(part 1 of 2)
# Autodesk Inventor assembly: Prototype II Assembly V3
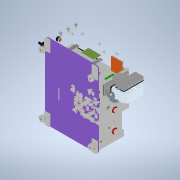
[picture p0: Inventor's stored thumbnail of the model, 180x180]
Saved by Autodesk Inventor 2021 (Build 250183000, 183)
## iProperties
Created: 2020-07-16
Part Number: Prototype II Assembly V3
Document SubType Name: Assembly
Designer: jgray
Author: jgray
## Documents named in this file (71)
- M:\Printed Electronics\Gas Sensors\Prototypes\Prototype II -Cartridge Reader V3\Prototype II Assembly V3.iam
- M:\Printed Electronics\Gas Sensors\Prototypes\Prototype II -Cartridge Reader V3\40ml Bottle and Lid.iam
- M:\Printed Electronics\Gas Sensors\Prototypes\Prototype II -Cartridge Reader V3\100ml Bottle and Lid.iam
- M:\Printed Electronics\Gas Sensors\Prototypes\Prototype II -Cartridge Reader V3\Full Cartridge Interface.iam
- M:\Printed Electronics\Gas Sensors\Prototypes\Prototype II -Cartridge Reader V3\Control & Sense Head PCB Assm.iam
- M:\Printed Electronics\Gas Sensors\Prototypes\Prototype II -Cartridge Reader V3\EC Sensor Sub-Assem.iam
- M:\Printed Electronics\Gas Sensors\Prototypes\Prototype II -Cartridge Reader V3\22Ah BatteryPack.ipt
- M:\Printed Electronics\Gas Sensors\Prototypes\Prototype II -Cartridge Reader V3\Battery Con.ipt
- M:\Printed Electronics\Gas Sensors\Prototypes\Prototype II -Cartridge Reader V3\Box Fixing Stud.ipt
- M:\Printed Electronics\Gas Sensors\Prototypes\Prototype II -Cartridge Reader V3\Coms Board V1.ipt
- M:\Printed Electronics\Gas Sensors\Prototypes\Prototype II -Cartridge Reader V3\Enclosure RS746-7396 body.ipt
- M:\Printed Electronics\Gas Sensors\Prototypes\Prototype II -Cartridge Reader V3\Internal Rear Plate.ipt
- M:\Printed Electronics\Gas Sensors\Prototypes\Prototype II -Cartridge Reader V3\Mechanical Driver Board.ipt
- M:\Printed Electronics\Gas Sensors\Prototypes\Prototype II -Cartridge Reader V3\Port Support Plate.ipt
- M:\Printed Electronics\Gas Sensors\Prototypes\Prototype II -Cartridge Reader V3\Right Bracket 50mm RS749-1680.ipt
- M:\Printed Electronics\Gas Sensors\Prototypes\Prototype II -Cartridge Reader V3\Status Indicator PCB.ipt
- M:\Printed Electronics\Gas Sensors\Prototypes\Prototype II -Cartridge Reader V3\Switch Mode PS PCB.ipt
- M:\Printed Electronics\Gas Sensors\Prototypes\Prototype II -Cartridge Reader V3\Top Divider.ipt
- M:\Printed Electronics\Gas Sensors\Prototypes\Prototype II -Cartridge Reader V3\Union Elbow 1-8 KQ2L01-00A SMC.ipt
- M:\Printed Electronics\Gas Sensors\Prototypes\Prototype II -Cartridge Reader V3\Vent Port M12.ipt
- M:\Printed Electronics\Gas Sensors\Prototypes\Prototype II -Cartridge Reader V3\Union Tee 1-8 KQ2T01-00A SMC.ipt
- M:\Printed Electronics\Gas Sensors\Prototypes\Prototype II -Cartridge Reader V3\Right Bracket 30mm RS749-1686.ipt
- M:\Printed Electronics\Gas Sensors\Prototypes\Prototype II -Cartridge Reader V3\Mounted Pump.iam
- M:\Printed Electronics\Gas Sensors\Prototypes\Prototype II -Cartridge Reader V3\Valve Assembly.iam
- M:\Printed Electronics\Gas Sensors\Prototypes\Prototype II -Cartridge Reader V3\Inner Top Plate.ipt
- M:\Printed Electronics\Gas Sensors\Prototypes\Prototype II -Cartridge Reader V3\Battery Side Plate.ipt
- M:\Printed Electronics\Gas Sensors\Prototypes\Prototype II -Cartridge Reader V3\LED Indicator Assem Farnell 1368996.iam
- M:\Printed Electronics\Gas Sensors\Prototypes\Prototype II -Cartridge Reader V3\Omron Switch DigiKey_Z6183-NDA22NS_2B[]_N[]A_G[]00_NN.iam
- M:\Printed Electronics\Gas Sensors\Prototypes\Prototype II -Cartridge Reader V3\Sprung Button Assm DigiKey EG5980-ND.iam
- M:\Printed Electronics\Gas Sensors\Prototypes\Prototype II -Cartridge Reader V3\Fixing Stud Pt 2.ipt
- M:\Printed Electronics\Gas Sensors\Prototypes\Prototype II -Cartridge Reader V3\Port Conversion Nut.ipt
- M:\Printed Electronics\Gas Sensors\Prototypes\Prototype II -Cartridge Reader V3\M8 Mudguard Washer RS 660-4771.ipt
- M:\Printed Electronics\Gas Sensors\Prototypes\Prototype II -Cartridge Reader V3\M12 Form B A2 Washer RS 530-810.ipt
- M:\Printed Electronics\Gas Sensors\Prototypes\Prototype II -Cartridge Reader V3\M12 Tap washer RS 530-270.ipt
- M:\Printed Electronics\Gas Sensors\Prototypes\Prototype II -Cartridge Reader V3\Cable Gland Lock Nut RS 822-9791.ipt
- M:\Printed Electronics\Gas Sensors\Prototypes\Prototype II -Cartridge Reader V3\SMC AS2002F Needle Valve RS 827-0755.ipt
- M:\Printed Electronics\Gas Sensors\Prototypes\Prototype II -Cartridge Reader V3\Battery Base Plate.ipt
- M:\Printed Electronics\Gas Sensors\Prototypes\Prototype II -Cartridge Reader V3\Internal Vert Divider.ipt
- M:\Printed Electronics\Gas Sensors\Prototypes\Prototype II -Cartridge Reader V3\SMC10-32UNF-1-8 KQ2H01-32N RS 840-4665.ipt
- M:\Printed Electronics\Gas Sensors\Prototypes\Prototype II -Cartridge Reader V3\Tube 1-8 5L.ipt
- M:\Printed Electronics\Gas Sensors\Prototypes\Prototype II -Cartridge Reader V3\SMC Elbow KQ2L23-04.ipt
- M:\Printed Electronics\Gas Sensors\Prototypes\Prototype II -Cartridge Reader V3\Legris4-4mm Elbow 31820400 RS 306-5993.ipt
- M:\Printed Electronics\Gas Sensors\Prototypes\Prototype II -Cartridge Reader V3\SMC Nipple 1-8to5-32 KQ2N01-03.ipt
- M:\Printed Electronics\Gas Sensors\Prototypes\Prototype II -Cartridge Reader V3\SMC 4mmMale-1-8Push KQ2R01-03(R23-04).ipt
- M:\Printed Electronics\Gas Sensors\Prototypes\Prototype II -Cartridge Reader V3\Bottle Base Plate.ipt
- M:\Printed Electronics\Gas Sensors\Prototypes\Prototype II -Cartridge Reader V3\Single Thrd Right Support Farnell1466883.ipt
- M:\Printed Electronics\Gas Sensors\Prototypes\Prototype II -Cartridge Reader V3\No Thrd Right Support Farnell1466881.ipt
- M:\Printed Electronics\Gas Sensors\Prototypes\Prototype II -Cartridge Reader V3\Cable Clip 3-1Dia RS817-8956.ipt
- M:\Printed Electronics\Gas Sensors\Prototypes\Prototype II -Cartridge Reader V3\Door Lock.ipt
- M:\Printed Electronics\Gas Sensors\Prototypes\Prototype II -Cartridge Reader V3\BAttery divider.ipt
- M:\Printed Electronics\Gas Sensors\Prototypes\Prototype II -Cartridge Reader V3\Bottle side plate.ipt
- M:\Printed Electronics\Gas Sensors\Prototypes\Prototype II -Cartridge Reader V3\Battery Top Plate.ipt
- C:\Users\jgray\Documents\Inventor\Content Center Files\R2021\en-US\BS 4320(2)\BS 4320 - M8 (Form B).ipt
- C:\Users\jgray\Documents\Inventor\Content Center Files\R2021\en-US\DIN 934\DIN 934 - M8 x 1.25.ipt
- M:\Printed Electronics\Gas Sensors\Prototypes\Prototype II -Cartridge Reader V3\Bottle Spacer Base.ipt
- M:\Printed Electronics\Gas Sensors\Prototypes\Prototype II -Cartridge Reader V3\Lower slide.ipt
- M:\Printed Electronics\Gas Sensors\Prototypes\Prototype II -Cartridge Reader V3\Upper slide.ipt
- M:\Printed Electronics\Gas Sensors\Prototypes\Prototype II -Cartridge Reader V3\Gas Side Top Cover.ipt
- M:\Printed Electronics\Gas Sensors\Prototypes\Prototype II -Cartridge Reader V3\Battery Cover.ipt
- M:\Printed Electronics\Gas Sensors\Prototypes\Prototype II -Cartridge Reader V3\Electronics cover.ipt
- M:\Printed Electronics\Gas Sensors\Prototypes\Prototype II -Cartridge Reader V3\corner spacers.ipt
- M:\Printed Electronics\Gas Sensors\Prototypes\Prototype II -Cartridge Reader V3\Silicone Seal washer.ipt
- M:\Printed Electronics\Gas Sensors\Prototypes\Prototype II -Cartridge Reader V3\Step-back spacer -electronics enc.ipt
- M:\Printed Electronics\Gas Sensors\Prototypes\Prototype II -Cartridge Reader V3\Step-back cover -electronics enc.ipt
- M:\Printed Electronics\Gas Sensors\Prototypes\Prototype II -Cartridge Reader V3\Top Bottle Front.ipt
- M:\Printed Electronics\Gas Sensors\Prototypes\Prototype II -Cartridge Reader V3\Top Bottle Middle.ipt
- M:\Printed Electronics\Gas Sensors\Prototypes\Prototype II -Cartridge Reader V3\Top Bottle Back.ipt
- M:\Printed Electronics\Gas Sensors\Prototypes\Prototype II -Cartridge Reader V3\upper plate slide.ipt
- M:\Printed Electronics\Gas Sensors\Prototypes\Prototype II -Cartridge Reader V3\LiPo cover.ipt
- M:\Printed Electronics\Gas Sensors\Prototypes\Prototype II -Cartridge Reader V3\Lipo Battery.ipt
- M:\Printed Electronics\Gas Sensors\Prototypes\Prototype II -Cartridge Reader V3\LipoBat Spacer.ipt
## Components (233 placed, 70 different names)
1. 40ml Bottle and Lid:1 [sub-assembly] — Angle:10, Mate:46, Mate:47, Mate:60, Mate:61, Flush:20, Flush:21, Flush:22
2. 40ml Bottle and Lid:2 [sub-assembly] — Angle:9, Mate:44, Mate:45, Mate:62, Mate:63, Flush:22
3. 40ml Bottle and Lid:3 [sub-assembly] — Angle:8, Mate:52, Mate:53, Mate:54, Mate:55, Flush:21
4. 40ml Bottle and Lid:4 [sub-assembly] — Angle:7, Mate:58, Flush:20, Flush:23, Mate:371
5. 100ml Bottle and Lid:1 [sub-assembly] — Angle:6, Mate:56, Flush:23, Mate:268
6. Full Cartridge Interface:1 [sub-assembly] — Mate:7, Mate:8, Mate:9, Mate:14, Mate:229, Mate:230, Mate:231, Mate:232, Flush:29, Mate:346, Flush:30
7. Control & Sense Head PCB Assm:1 [sub-assembly] — Flush:29, Mate:346, Flush:30
8. EC Sensor Sub-Assem:1 [sub-assembly] — Angle:1, Angle:2, Mate:12, Flush:8
9. 22Ah BatteryPack:1 — Mate:2, Mate:67, Flush:14, Mate:415, Mate:416, Mate:417
10. 22Ah BatteryPack:2 — Mate:1, Flush:14, Mate:145, Mate:383, Mate:622
11. Battery Con:1 — Mate:622
12. Battery Con:2 — Mate:415, Angle:66, Mate:416, Mate:417
13. Box Fixing Stud:1 — Mate:31, Mate:32, Mate:97, Mate:98, Mate:521, Mate:527, Mate:614
14. Box Fixing Stud:2 — Mate:35, Flush:11, Mate:102, Mate:517, Mate:525, Mate:610, Mate:615
15. Box Fixing Stud:3 — Mate:36, Flush:10, Mate:99, Mate:101, Angle:67, Mate:513, Mate:514, Mate:612, Mate:616
16. Box Fixing Stud:4 — Mate:33, Mate:34, Flush:10, Flush:11, Mate:6, Mate:100, Mate:519, Mate:526, Mate:619
17. Coms Board V1:1 — Mate:629, Mate:630, Mate:631, Mate:636, Mate:637, Mate:675
18. Enclosure RS746-7396 body:1 — Mate:5, Mate:7, Mate:8, Mate:9, Mate:13, Mate:15, Mate:31, Mate:32, Mate:33, Mate:34, Mate:35, Mate:36, Mate:78, Mate:79, Mate:80, Mate:81, Mate:82, Mate:83, Mate:84, Mate:85, Mate:86, Mate:87, Mate:88, Mate:89, Mate:90, Flush:15, Mate:91, Mate:92, Mate:94, Mate:96, Mate:105, Mate:106, Mate:107, Mate:108, Mate:113, Mate:114, Mate:122, Tangent:1, Tangent:2, Tangent:3, Tangent:4
19. Internal Rear Plate:1 — Mate:1, Mate:2, Mate:5, Mate:6, Angle:1, Angle:2, Mate:12, Angle:3, Angle:4, Flush:8, Mate:22, Angle:5, Mate:24, Flush:9, Mate:25, Mate:26, Mate:27, Mate:28, Mate:29, Mate:30, Mate:41, Mate:43, Mate:65, Mate:72, Mate:74, Mate:124, Mate:125, Mate:126, Mate:127, Mate:128, Mate:129, Mate:130, Mate:133, Mate:139, Mate:140, Mate:141, Angle:16, Angle:17, Angle:18, Angle:21, Mate:174, Angle:22, Angle:24, Mate:177, Mate:178, Mate:182, Mate:183, Angle:27, Angle:29, Mate:186, Mate:191, Mate:196, Mate:197, Mate:199, Angle:35, Angle:36, Angle:38, Mate:210, Mate:69, Mate:221, Mate:222, Mate:224, Mate:227, Angle:48, Mate:235, Mate:238, Angle:53, Mate:257, Mate:269, Mate:270, Mate:273, Mate:274, Angle:56, Angle:57, Angle:58, Mate:292, Mate:313, Mate:314, Mate:340, Mate:341, Mate:342, Mate:343, Mate:344, Mate:348, Mate:349, Mate:350, Mate:352, Mate:353, Mate:354, Mate:364, Angle:60, Angle:61, Angle:62, Angle:63, Angle:64, Angle:65, Mate:386, Mate:392, Mate:393, Mate:394, Mate:412, Mate:414, Mate:423, Mate:446, Mate:449, Mate:465, Mate:467, Mate:468, Mate:469, Mate:470, Mate:486, Mate:487, Mate:500, Mate:502, Mate:507, Mate:511, Mate:512, Mate:516, Mate:518, Mate:520, Mate:528, Mate:607, Mate:609, Mate:611, Angle:80, Mate:613, Angle:81, Mate:648, Mate:661, Mate:664
20. Mechanical Driver Board:1 — Mate:375, Mate:378, Mate:379
21. Port Support Plate:1 — Mate:13, Mate:14, Mate:15, Mate:16, Mate:17, Mate:18, Mate:19, Mate:20, Mate:21, Mate:70, Flush:31, Mate:375, Mate:378, Mate:379
22. Right Bracket 50mm RS749-1680:1 — Mate:25, Mate:26, Mate:27, Mate:75, Mate:77
23. Right Bracket 50mm RS749-1680:2 — Mate:28, Mate:29, Mate:30, Mate:76
24. Right Bracket 50mm RS749-1680:3 — Mate:72, Mate:73, Mate:74
25. Right Bracket 50mm RS749-1680:4 — Mate:16, Mate:18, Mate:19, Mate:23
26. Right Bracket 50mm RS749-1680:5 — Mate:17, Mate:20, Mate:21
27. Status Indicator PCB:1 — Mate:670, Mate:671, Mate:672
28. Switch Mode PS PCB:1 — Mate:22, Angle:5, Mate:344
29. Top Divider:1 — Mate:23, Mate:24, Flush:9, Mate:40, Flush:13, Mate:66, Mate:73, Angle:14, Angle:45, Angle:46, Angle:47, Mate:233, Mate:244, Mate:374, Mate:376, Mate:377, Mate:388, Mate:389, Mate:390, Mate:397, Mate:399, Mate:418, Mate:421, Mate:551, Flush:33, Flush:34, Mate:553, Mate:554, Mate:556, Mate:557, Mate:580, Mate:581, Flush:45, Flush:46, Mate:583, Mate:584, Mate:591, Mate:592, Angle:72, Angle:73, Angle:74, Angle:75, Mate:594, Mate:595, Mate:596, Mate:603, Mate:604, Mate:605, Angle:77, Angle:78, Angle:79, Mate:632, Mate:633, Mate:634, Mate:635, Mate:673, Mate:676, Mate:678, Mate:679, Mate:680, Mate:681
30. Union Elbow 1-8 KQ2L01-00A SMC:1 — Angle:22, Mate:182, Mate:185, Flush:24, Angle:27, Mate:192, Mate:194, Mate:322, Mate:323
31. Vent Port M12:1 — Mate:78, Mate:82, Mate:103, Mate:116
32. Union Elbow 1-8 KQ2L01-00A SMC:2 — Mate:178, Mate:337, Mate:338, Mate:339
33. Vent Port M12:2 — Mate:79, Mate:81, Mate:123
34. Union Elbow 1-8 KQ2L01-00A SMC:3 — Flush:16, Angle:18
35. Union Elbow 1-8 KQ2L01-00A SMC:4 — Mate:56, Flush:16, Mate:211
36. Union Elbow 1-8 KQ2L01-00A SMC:5 — Mate:53, Mate:55, Flush:18, Mate:184, Angle:28, Angle:32
37. Union Elbow 1-8 KQ2L01-00A SMC:6 — Mate:52, Mate:54, Flush:18, Angle:16, Mate:181
38. Union Elbow 1-8 KQ2L01-00A SMC:7 — Mate:223, Angle:60, Mate:371
39. Union Elbow 1-8 KQ2L01-00A SMC:8 — Mate:58, Mate:372
40. Union Elbow 1-8 KQ2L01-00A SMC:9 — Mate:46, Mate:61, Angle:23, Mate:176, Mate:256
41. Union Elbow 1-8 KQ2L01-00A SMC:10 — Mate:47, Mate:60, Mate:187, Mate:370
42. Union Elbow 1-8 KQ2L01-00A SMC:11 — Mate:45, Mate:62, Flush:17, Mate:337
43. Union Elbow 1-8 KQ2L01-00A SMC:12 — Mate:44, Mate:63, Flush:17, Angle:17, Mate:185
44. Union Tee 1-8 KQ2T01-00A SMC:1 — Mate:239, Mate:240, Angle:50, Mate:241, Angle:55, Mate:313, Mate:353
45. Union Tee 1-8 KQ2T01-00A SMC:2 — Angle:29, Mate:186, Mate:187, Mate:189, Mate:190, Mate:204, Mate:332, Mate:333, Angle:64, Mate:370
46. Union Tee 1-8 KQ2T01-00A SMC:3 — Angle:21, Mate:174, Mate:181, Mate:204, Angle:38, Mate:330, Mate:334
47. Right Bracket 30mm RS749-1686:2 — Mate:408, Mate:409, Mate:410, Mate:411
48. Right Bracket 30mm RS749-1686:3 — Mate:404, Mate:405, Mate:406, Mate:407
49. Right Bracket 30mm RS749-1686:4 — Mate:401, Mate:402, Mate:403
50. Right Bracket 30mm RS749-1686:5 — Mate:397, Mate:398, Mate:399, Mate:400
51. Right Bracket 30mm RS749-1686:6 — Mate:388, Mate:389, Mate:390, Mate:391
52. Right Bracket 30mm RS749-1686:8 — Mate:253, Mate:254, Mate:255, Angle:54
53. Mounted Pump:1 [sub-assembly] — Mate:70, Flush:31, Mate:374
54. Valve Assembly:1 [sub-assembly] — Mate:69, Angle:40, Mate:342
55. Valve Assembly:2 [sub-assembly] — Mate:196, Angle:34, Mate:340
56. Valve Assembly:3 [sub-assembly] — Mate:191, Angle:32, Angle:34, Angle:40, Mate:341
57. Inner Top Plate:1 — Mate:75, Mate:76, Mate:77, Mate:598, Mate:599, Mate:623, Mate:624, Mate:625, Mate:626, Mate:627, Mate:667, Mate:668, Mate:669, Mate:670, Mate:671, Mate:672
58. Right Bracket 50mm RS749-1680:8 — Mate:40, Mate:41, Mate:43
59. Battery Side Plate:1 — Mate:65, Flush:13, Mate:66, Mate:67, Mate:131, Mate:132, Mate:134, Mate:135, Mate:404, Mate:406, Mate:419, Mate:420, Mate:464, Mate:471, Mate:490, Mate:558, Mate:574, Mate:575, Flush:42, Mate:579, Flush:47
60. Vent Port M12:3 — Mate:80, Mate:83, Mate:104, Mate:115, Mate:119
61. LED Indicator Assem Farnell 1368996:1 [sub-assembly] — Mate:84, Mate:89
62. LED Indicator Assem Farnell 1368996:2 [sub-assembly] — Mate:86, Mate:87
63. LED Indicator Assem Farnell 1368996:3 [sub-assembly] — Mate:85, Mate:88
64. Omron Switch DigiKey_Z6183-NDA22NS_2B[]_N[]A_G[]00_NN:1 [sub-assembly] — Mate:90, Flush:15, Angle:14
65. Sprung Button Assm DigiKey EG5980-ND:1 [sub-assembly] — Mate:91, Mate:92
66. Fixing Stud Pt 2:1 — Mate:94, Mate:100, Mate:111, Mate:608, Mate:620
67. Fixing Stud Pt 2:2 — Mate:99, Mate:101, Mate:109, Mate:618
68. Fixing Stud Pt 2:3 — Mate:96, Mate:102, Mate:110, Mate:617
69. Fixing Stud Pt 2:4 — Mate:97, Mate:98, Mate:112, Mate:621
70. Port Conversion Nut:1 — Mate:103, Mate:121, Mate:157, Mate:159, Mate:160
71. Port Conversion Nut:2 — Mate:104, Mate:120, Mate:158, Mate:161
72. M8 Mudguard Washer RS 660-4771:1 — Mate:107, Mate:112
73. M8 Mudguard Washer RS 660-4771:2 — Mate:105, Mate:111
74. M8 Mudguard Washer RS 660-4771:3 — Mate:108, Mate:109
75. M8 Mudguard Washer RS 660-4771:4 — Mate:106, Mate:110
76. M12 Form B A2 Washer RS 530-810:1 — Mate:117, Mate:121, Mate:157
77. M12 Tap washer RS 530-270:1 — Mate:113, Mate:116, Mate:117
78. M12 Form B A2 Washer RS 530-810:2 — Mate:118, Mate:119, Mate:120
79. M12 Tap washer RS 530-270:2 — Mate:114, Mate:115, Mate:118
80. Cable Gland Lock Nut RS 822-9791:1 — Mate:122, Mate:123
81. Right Bracket 50mm RS749-1680:9 — Mate:133, Mate:134, Mate:135
82. Right Bracket 50mm RS749-1680:10 — Mate:130, Mate:131, Mate:132
83. Right Bracket 50mm RS749-1680:12 — Mate:392, Mate:393, Mate:394, Mate:395, Mate:396
84. Right Bracket 50mm RS749-1680:13 — Mate:139, Mate:140, Mate:141, Mate:142, Mate:143, Mate:144
85. SMC AS2002F Needle Valve RS 827-0755:1 — Mate:244, Mate:246, Flush:28, Mate:248, Mate:252, Mate:376, Mate:377
86. Right Bracket 50mm RS749-1680:14 — Mate:125, Mate:128, Mate:129, Mate:137, Mate:138
87. Right Bracket 50mm RS749-1680:15 — Mate:507, Mate:508, Mate:509, Mate:510, Mate:511
88. Right Bracket 50mm RS749-1680:17 — Mate:124, Mate:126, Mate:127, Mate:136
89. Battery Base Plate:1 — Mate:136, Mate:137, Mate:138, Mate:145, Mate:384, Mate:385, Mate:401, Mate:403, Mate:405, Mate:407, Mate:408, Mate:411, Mate:564, Mate:565, Mate:566, Mate:567, Mate:569, Mate:570, Mate:571, Mate:572, Flush:37, Flush:38, Flush:39, Flush:40
90. Internal Vert Divider:1 — Mate:142, Mate:143, Mate:144, Mate:255, Mate:258, Mate:271, Mate:272, Mate:383, Mate:387, Mate:391, Mate:409, Mate:410, Mate:413, Mate:459, Mate:461, Mate:462, Mate:497, Mate:498, Mate:505, Mate:506, Mate:529, Mate:531, Mate:533, Mate:539, Mate:540, Mate:541, Mate:548, Mate:549, Flush:35, Mate:561, Mate:562, Mate:573, Flush:36, Mate:577, Mate:585, Mate:586, Mate:587, Mate:588, Mate:589, Mate:590, Mate:647, Mate:662, Mate:665, Mate:666, Mate:677
91. SMC10-32UNF-1-8 KQ2H01-32N RS 840-4665:1 — Mate:159, Mate:160, Mate:163, Mate:164, Mate:251
92. SMC10-32UNF-1-8 KQ2H01-32N RS 840-4665:2 — Mate:158, Mate:161, Mate:345
93. Tube 1-8 5L:2 — Mate:163, Mate:164
94. Union Elbow 1-8 KQ2L01-00A SMC:14 — Mate:171, Angle:23, Angle:24, Mate:176, Mate:256
95. Union Elbow 1-8 KQ2L01-00A SMC:15 — Mate:171, Mate:345
96. Union Elbow 1-8 KQ2L01-00A SMC:16 — Mate:189, Mate:190, Mate:209
97. Union Elbow 1-8 KQ2L01-00A SMC:17 — Mate:197, Mate:201, Angle:35, Angle:39, Mate:315, Mate:316, Mate:348, Angle:63, Angle:65
98. Union Elbow 1-8 KQ2L01-00A SMC:18 — Mate:177, Mate:192, Mate:194, Mate:309, Mate:310
99. Union Elbow 1-8 KQ2L01-00A SMC:19 — Mate:199, Mate:202, Mate:203, Angle:49, Mate:295, Mate:296, Mate:350
100. Union Elbow 1-8 KQ2L01-00A SMC:20 — Mate:183, Mate:184, Flush:24, Angle:28, Mate:193, Mate:195, Flush:25, Angle:44
101. Union Elbow 1-8 KQ2L01-00A SMC:21 — Mate:193, Mate:195, Flush:25, Mate:318, Mate:319
102. Union Elbow 1-8 KQ2L01-00A SMC:22 — Mate:201, Mate:202, Mate:203, Angle:36, Angle:37, Mate:207, Mate:354
103. Union Elbow 1-8 KQ2L01-00A SMC:23 — Mate:210, Mate:211, Angle:39, Mate:277, Mate:328, Mate:329, Mate:349
104. Union Elbow 1-8 KQ2L01-00A SMC:24 — Mate:208, Mate:209
105. Union Elbow 1-8 KQ2L01-00A SMC:26 — Angle:37, Mate:207, Mate:208, Mate:290, Mate:291, Mate:292
106. Union Elbow 1-8 KQ2L01-00A SMC:28 — Mate:221, Mate:226, Angle:53, Angle:55, Mate:282, Mate:283, Mate:284, Mate:285
107. Union Elbow 1-8 KQ2L01-00A SMC:29 — Mate:222, Mate:223, Mate:226, Angle:44, Angle:51, Mate:326, Mate:327, Mate:364, Angle:62
108. Union Elbow 1-8 KQ2L01-00A SMC:30 — Mate:224, Angle:50, Angle:51, Mate:314, Mate:324, Mate:325, Angle:61, Mate:372
109. Union Elbow 1-8 KQ2L01-00A SMC:31 — Mate:227, Mate:277, Mate:303, Mate:304, Mate:305, Mate:306, Mate:343
110. Union Elbow 1-8 KQ2L01-00A SMC:32 — Mate:251, Mate:253, Mate:254, Angle:54
111. SMC Elbow KQ2L23-04:2 — Mate:248, Mate:252
112. Legris4-4mm Elbow 31820400 RS 306-5993:1 — Mate:231, Mate:232, Angle:45, Mate:243, Flush:27
113. Legris4-4mm Elbow 31820400 RS 306-5993:2 — Mate:229, Mate:230, Angle:46, Mate:234, Mate:242, Flush:26
114. Union Elbow 1-8 KQ2L01-00A SMC:33 — Mate:235, Mate:236, Angle:49, Mate:241, Mate:299, Mate:300, Mate:301, Mate:302
115. Union Elbow 1-8 KQ2L01-00A SMC:34 — Angle:47, Angle:48, Mate:233, Mate:234, Mate:236
116. Union Elbow 1-8 KQ2L01-00A SMC:35 — Mate:238, Mate:239, Mate:240, Mate:278, Mate:279, Mate:280, Mate:281
117. SMC Nipple 1-8to5-32 KQ2N01-03:1 — Mate:243, Flush:27
118. SMC Nipple 1-8to5-32 KQ2N01-03:2 — Mate:246, Flush:28
119. SMC 4mmMale-1-8Push KQ2R01-03(R23-04):2 — Mate:242, Flush:26
120. Bottle Base Plate:1 — Mate:257, Mate:258, Mate:268, Mate:275, Mate:276, Mate:422, Mate:424, Flush:32, Mate:450, Mate:451, Mate:453, Mate:454, Mate:456, Mate:457, Mate:458, Mate:460, Mate:463, Angle:67, Mate:530, Mate:532, Mate:535
121. Single Thrd Right Support Farnell1466883:8 — Mate:565, Mate:571, Flush:38
122. No Thrd Right Support Farnell1466881:1 — Mate:269, Mate:273, Mate:275
123. No Thrd Right Support Farnell1466881:2 — Mate:270, Mate:274, Mate:276
124. No Thrd Right Support Farnell1466881:3 — Mate:271, Mate:387
125. No Thrd Right Support Farnell1466881:4 — Mate:448, Mate:454, Mate:455, Mate:457
126. No Thrd Right Support Farnell1466881:5 — Mate:447, Mate:452, Mate:453, Mate:456
127. No Thrd Right Support Farnell1466881:6 — Mate:446, Mate:449, Mate:450, Mate:451
128. No Thrd Right Support Farnell1466881:7 — Mate:468, Mate:496, Mate:501, Mate:502
129. No Thrd Right Support Farnell1466881:8 — Mate:470, Mate:479, Mate:485, Mate:486
130. No Thrd Right Support Farnell1466881:9 — Mate:272, Mate:422, Mate:458, Mate:459
131. No Thrd Right Support Farnell1466881:11 — Mate:469, Mate:478, Mate:487, Mate:488
132. No Thrd Right Support Farnell1466881:12 — Mate:467, Mate:495, Mate:499, Mate:500
133. Cable Clip 3-1Dia RS817-8956:2 — Angle:56, Mate:278, Mate:281
134. Cable Clip 3-1Dia RS817-8956:3 — Angle:58, Mate:330, Mate:334
135. Cable Clip 3-1Dia RS817-8956:4 — Angle:57, Mate:279, Mate:280
136. Cable Clip 3-1Dia RS817-8956:5 — Mate:282, Mate:285
137. Cable Clip 3-1Dia RS817-8956:6 — Mate:283, Mate:284
138. Cable Clip 3-1Dia RS817-8956:9 — Mate:290, Mate:291
139. Cable Clip 3-1Dia RS817-8956:12 — Mate:295, Mate:296
140. Cable Clip 3-1Dia RS817-8956:13 — Mate:299, Mate:300
141. Cable Clip 3-1Dia RS817-8956:14 — Mate:301, Mate:302
142. Cable Clip 3-1Dia RS817-8956:15 — Mate:303, Mate:304
143. Cable Clip 3-1Dia RS817-8956:16 — Mate:305, Mate:306
144. Cable Clip 3-1Dia RS817-8956:19 — Mate:322, Mate:323
145. Cable Clip 3-1Dia RS817-8956:20 — Mate:328, Mate:329, Mate:352
146. Cable Clip 3-1Dia RS817-8956:22 — Mate:309, Mate:310
147. Cable Clip 3-1Dia RS817-8956:24 — Mate:318, Mate:319
148. Cable Clip 3-1Dia RS817-8956:25 — Mate:315, Mate:316
149. Cable Clip 3-1Dia RS817-8956:26 — Mate:324, Mate:325
150. Cable Clip 3-1Dia RS817-8956:27 — Mate:326, Mate:327
151. Cable Clip 3-1Dia RS817-8956:29 — Mate:332, Mate:333
152. Cable Clip 3-1Dia RS817-8956:30 — Mate:338, Mate:339
153. Door Lock:1 — Tangent:3, Tangent:4
154. Door Lock:2 — Tangent:1, Tangent:2
155. BAttery divider:1 — Mate:384, Mate:385, Mate:386, Mate:395, Mate:396, Mate:398, Mate:400, Mate:402, Angle:66, Mate:466, Mate:480, Mate:481, Mate:484, Mate:491, Mate:493, Mate:494, Mate:563, Mate:568, Flush:41
156. Right Bracket 30mm RS749-1686:9 — Mate:412, Mate:413, Mate:414
157. Right Bracket 30mm RS749-1686:10 — Mate:418, Mate:419, Mate:420, Mate:421
158. Bottle side plate:1 — Mate:423, Mate:424, Flush:32, Mate:447, Mate:448, Mate:452, Mate:455, Mate:508, Mate:509, Mate:510, Mate:536, Mate:537, Mate:538, Mate:542, Mate:543, Mate:544, Mate:545, Mate:546, Mate:552, Mate:582, Mate:593, Angle:71, Mate:650, Mate:654, Mate:659
159. Single Thrd Right Support Farnell1466883:9 — Mate:548, Mate:549, Angle:69, Mate:550
160. Single Thrd Right Support Farnell1466883:10 — Mate:557, Mate:580, Flush:46
161. Single Thrd Right Support Farnell1466883:13 — Mate:545, Mate:546, Angle:68, Mate:547
162. Single Thrd Right Support Farnell1466883:15 — Mate:556, Mate:581, Flush:45
163. Single Thrd Right Support Farnell1466883:16 — Mate:558, Mate:579, Flush:47
164. Single Thrd Right Support Farnell1466883:17 — Mate:559, Mate:578, Flush:44
165. Single Thrd Right Support Farnell1466883:18 — Mate:560, Mate:576, Flush:43
166. Single Thrd Right Support Farnell1466883:19 — Mate:561, Mate:577, Angle:70
167. No Thrd Right Support Farnell1466881:13 — Mate:460, Mate:461, Mate:462, Mate:463
168. Battery Top Plate:1 — Mate:464, Mate:465, Mate:466, Mate:472, Mate:473, Mate:474, Mate:475, Mate:476, Mate:477, Mate:478, Mate:479, Mate:482, Mate:483, Mate:485, Mate:488, Mate:489, Mate:492, Mate:495, Mate:496, Mate:499, Mate:501, Mate:503, Mate:504, Mate:559, Mate:560, Mate:576, Mate:578, Flush:43, Flush:44, Angle:70
169. No Thrd Right Support Farnell1466881:16 — Mate:476, Mate:498, Mate:504, Mate:505
170. No Thrd Right Support Farnell1466881:17 — Mate:474, Mate:492, Mate:493, Mate:494
171. No Thrd Right Support Farnell1466881:18 — Mate:473, Mate:481, Mate:482, Mate:491
172. No Thrd Right Support Farnell1466881:19 — Mate:471, Mate:477, Mate:489, Mate:490
173. No Thrd Right Support Farnell1466881:20 — Mate:472, Mate:480, Mate:483, Mate:484
174. No Thrd Right Support Farnell1466881:21 — Mate:475, Mate:497, Mate:503, Mate:506
175. BS 4320 Form AB M8 (Form B):1 — Mate:512, Mate:513, Mate:515
176. BS 4320 Form AB M8 (Form B):2 — Mate:516, Mate:517, Mate:524
177. BS 4320 Form AB M8 (Form B):3 — Mate:520, Mate:521, Mate:522
178. BS 4320 Form AB M8 (Form B):4 — Mate:518, Mate:519, Mate:523
179. DIN 934 - replaced by DIN EN 24032/28673/28674 M8:1 — Mate:524, Mate:525
180. DIN 934 - replaced by DIN EN 24032/28673/28674 M8:2 — Mate:514, Mate:515
181. DIN 934 - replaced by DIN EN 24032/28673/28674 M8:3 — Mate:522, Mate:527
182. DIN 934 - replaced by DIN EN 24032/28673/28674 M8:4 — Mate:523, Mate:526
183. Bottle Spacer Base:1 — Mate:528, Mate:529, Mate:530, Angle:68, Mate:547, Angle:69, Mate:550
184. Lower slide:1 — Mate:535, Mate:536, Mate:537, Mate:538
185. Lower slide:2 — Mate:531, Mate:532, Mate:533, Mate:677
186. Upper slide:1 — Mate:542, Mate:543, Mate:544, Mate:646, Mate:655, Mate:658
187. Upper slide:2 — Mate:539, Mate:540, Mate:541, Mate:649, Mate:652, Mate:656, Mate:657
188. Gas Side Top Cover:1 — Mate:551, Mate:552, Flush:33
189. Battery Cover:1 — Flush:34, Flush:35, Mate:553
190. Electronics cover:1 — Mate:554, Mate:638, Mate:639, Mate:640, Mate:641, Mate:642
191. Single Thrd Right Support Farnell1466883:20 — Mate:563, Mate:568, Flush:41
192. Single Thrd Right Support Farnell1466883:21 — Mate:564, Mate:572, Flush:37
193. Single Thrd Right Support Farnell1466883:22 — Mate:567, Mate:570, Flush:40
194. Single Thrd Right Support Farnell1466883:23 — Mate:586, Mate:589, Angle:75, Angle:76
195. Single Thrd Right Support Farnell1466883:24 — Mate:587, Mate:588, Angle:76
196. Single Thrd Right Support Farnell1466883:25 — Mate:562, Mate:573, Flush:36
197. Single Thrd Right Support Farnell1466883:26 — Mate:566, Mate:569, Flush:39
198. Single Thrd Right Support Farnell1466883:27 — Mate:582, Mate:593, Angle:71
199. Single Thrd Right Support Farnell1466883:28 — Mate:583, Mate:592, Angle:72
200. Single Thrd Right Support Farnell1466883:29 — Mate:584, Mate:591, Angle:73
201. Single Thrd Right Support Farnell1466883:31 — Mate:585, Mate:590, Angle:74
202. Single Thrd Right Support Farnell1466883:32 — Mate:574, Mate:575, Flush:42
203. Single Thrd Right Support Farnell1466883:33 — Mate:594, Mate:603, Angle:79, Mate:638, Mate:639
204. Single Thrd Right Support Farnell1466883:34 — Mate:595, Mate:604, Angle:78
205. Single Thrd Right Support Farnell1466883:35 — Mate:599, Mate:667
206. Single Thrd Right Support Farnell1466883:36 — Mate:596, Mate:605, Angle:77
207. Single Thrd Right Support Farnell1466883:37 — Mate:598, Mate:669
208. corner spacers:1 — Mate:613, Mate:614, Angle:81
209. corner spacers:2 — Mate:611, Mate:612, Angle:80
210. corner spacers:3 — Mate:609, Mate:610
211. corner spacers:4 — Mate:607, Mate:608
212. Silicone Seal washer:1 — Mate:621
213. Silicone Seal washer:2 — Mate:619, Mate:620
214. Silicone Seal washer:3 — Mate:615, Mate:617
215. Silicone Seal washer:4 — Mate:616, Mate:618
216. Single Thrd Right Support Farnell1466883:38 — Mate:625, Mate:626, Mate:630
217. Single Thrd Right Support Farnell1466883:39 — Mate:632, Mate:633, Mate:636, Mate:675
218. Single Thrd Right Support Farnell1466883:40 — Mate:627, Mate:668
219. Single Thrd Right Support Farnell1466883:41 — Mate:623, Mate:624, Mate:629, Mate:631
220. Single Thrd Right Support Farnell1466883:42 — Mate:634, Mate:635, Mate:637
221. Step-back spacer -electronics enc:1 — Mate:640, Mate:641, Mate:642, Mate:643, Mate:644, Mate:645
222. Step-back cover -electronics enc:1 — Mate:643, Mate:644, Mate:645
223. Top Bottle Front:1 — Mate:652, Mate:653, Mate:654, Angle:82, Angle:83
224. Top Bottle Middle:1 — Mate:649, Mate:650, Mate:651, Mate:653, Mate:660, Mate:663
225. Top Bottle Back:1 — Mate:646, Mate:647, Mate:648, Mate:651
226. Single Thrd Right Support Farnell1466883:43 — Mate:655, Mate:658, Angle:82
227. Single Thrd Right Support Farnell1466883:44 — Mate:656, Mate:657, Angle:83
228. upper plate slide:1 — Mate:659, Mate:660, Mate:661
229. upper plate slide:2 — Mate:662, Mate:663, Mate:664, Mate:665, Mate:666
230. LiPo cover:1 — Mate:673, Flush:48
231. Lipo Battery:1 — Mate:676, Flush:48
232. LipoBat Spacer:1 — Mate:679, Mate:680, Mate:681, Mate:682, Flush:50
233. LipoBat Spacer:2 — Mate:678, Mate:682, Flush:50
## Relationships (653: Mate 542, Angle 67, Flush 40, Tangent 4)
- Mate:1: 22Ah BatteryPack:2 ↔ Internal Rear Plate:1
- Mate:2: 22Ah BatteryPack:1 ↔ Internal Rear Plate:1
- Mate:5 (0.6 mm): Enclosure RS746-7396 body:1 ↔ Internal Rear Plate:1
- Mate:6: Box Fixing Stud:4 ↔ Internal Rear Plate:1
- Mate:7: Full Cartridge Interface:1 ↔ Enclosure RS746-7396 body:1
- Mate:8: Full Cartridge Interface:1 ↔ Enclosure RS746-7396 body:1
- Mate:9: Full Cartridge Interface:1 ↔ Enclosure RS746-7396 body:1
- Angle:1 (180 deg): EC Sensor Sub-Assem:1 ↔ Internal Rear Plate:1
- Angle:2 (0 deg): EC Sensor Sub-Assem:1 ↔ Internal Rear Plate:1
- Mate:12 (2 mm): EC Sensor Sub-Assem:1 ↔ Internal Rear Plate:1
- Angle:3 (180 deg): Internal Rear Plate:1
- Angle:4 (180 deg): Internal Rear Plate:1
- Flush:8 (40 mm): EC Sensor Sub-Assem:1 ↔ Internal Rear Plate:1
- Mate:13: Enclosure RS746-7396 body:1 ↔ Port Support Plate:1
- Mate:14: Full Cartridge Interface:1 ↔ Port Support Plate:1
- Mate:15: Enclosure RS746-7396 body:1 ↔ Port Support Plate:1
- Mate:16: Port Support Plate:1 ↔ Right Bracket 50mm RS749-1680:4
- Mate:17: Port Support Plate:1 ↔ Right Bracket 50mm RS749-1680:5
- Mate:18: Port Support Plate:1 ↔ Right Bracket 50mm RS749-1680:4
- Mate:19: Port Support Plate:1 ↔ Right Bracket 50mm RS749-1680:4
- Mate:20: Port Support Plate:1 ↔ Right Bracket 50mm RS749-1680:5
- Mate:21: Port Support Plate:1 ↔ Right Bracket 50mm RS749-1680:5
- Mate:22 (8 mm): Internal Rear Plate:1 ↔ Switch Mode PS PCB:1
- Angle:5 (90 deg): Internal Rear Plate:1 ↔ Switch Mode PS PCB:1
- Angle:6 (0 deg): 100ml Bottle and Lid:1
- Angle:7 (0 deg): 40ml Bottle and Lid:4
- Angle:8 (0 deg): 40ml Bottle and Lid:3
- Angle:9 (0 deg): 40ml Bottle and Lid:2
- Angle:10 (0 deg): 40ml Bottle and Lid:1
- Mate:23: Right Bracket 50mm RS749-1680:4 ↔ Top Divider:1
- Mate:24: Internal Rear Plate:1 ↔ Top Divider:1
- Flush:9: Internal Rear Plate:1 ↔ Top Divider:1
- Mate:25: Internal Rear Plate:1 ↔ Right Bracket 50mm RS749-1680:1
- Mate:26: Internal Rear Plate:1 ↔ Right Bracket 50mm RS749-1680:1
- Mate:27: Internal Rear Plate:1 ↔ Right Bracket 50mm RS749-1680:1
- Mate:28: Internal Rear Plate:1 ↔ Right Bracket 50mm RS749-1680:2
- Mate:29: Internal Rear Plate:1 ↔ Right Bracket 50mm RS749-1680:2
- Mate:30: Internal Rear Plate:1 ↔ Right Bracket 50mm RS749-1680:2
- Mate:31: Box Fixing Stud:1 ↔ Enclosure RS746-7396 body:1
- Mate:32 (1 mm): Box Fixing Stud:1 ↔ Enclosure RS746-7396 body:1
- Mate:33: Box Fixing Stud:4 ↔ Enclosure RS746-7396 body:1
- Mate:34 (1 mm): Box Fixing Stud:4 ↔ Enclosure RS746-7396 body:1
- Mate:35: Box Fixing Stud:2 ↔ Enclosure RS746-7396 body:1
- Mate:36: Box Fixing Stud:3 ↔ Enclosure RS746-7396 body:1
- Flush:10: Box Fixing Stud:3 ↔ Box Fixing Stud:4
- Flush:11: Box Fixing Stud:2 ↔ Box Fixing Stud:4
- Mate:40: Top Divider:1 ↔ Right Bracket 50mm RS749-1680:8
- Mate:41: Internal Rear Plate:1 ↔ Right Bracket 50mm RS749-1680:8
- Mate:43: Internal Rear Plate:1 ↔ Right Bracket 50mm RS749-1680:8
- Mate:44 (8 mm): 40ml Bottle and Lid:2 ↔ Union Elbow 1-8 KQ2L01-00A SMC:12
- Mate:45: 40ml Bottle and Lid:2 ↔ Union Elbow 1-8 KQ2L01-00A SMC:11
- Mate:46: 40ml Bottle and Lid:1 ↔ Union Elbow 1-8 KQ2L01-00A SMC:9
- Mate:47: 40ml Bottle and Lid:1 ↔ Union Elbow 1-8 KQ2L01-00A SMC:10
- Mate:52: 40ml Bottle and Lid:3 ↔ Union Elbow 1-8 KQ2L01-00A SMC:6
- Mate:53 (8 mm): 40ml Bottle and Lid:3 ↔ Union Elbow 1-8 KQ2L01-00A SMC:5
- Mate:54: 40ml Bottle and Lid:3 ↔ Union Elbow 1-8 KQ2L01-00A SMC:6
- Mate:55: 40ml Bottle and Lid:3 ↔ Union Elbow 1-8 KQ2L01-00A SMC:5
- Mate:56: 100ml Bottle and Lid:1 ↔ Union Elbow 1-8 KQ2L01-00A SMC:4
- Mate:58: 40ml Bottle and Lid:4 ↔ Union Elbow 1-8 KQ2L01-00A SMC:8
- Mate:60: 40ml Bottle and Lid:1 ↔ Union Elbow 1-8 KQ2L01-00A SMC:10
- Mate:61: 40ml Bottle and Lid:1 ↔ Union Elbow 1-8 KQ2L01-00A SMC:9
- Mate:62: 40ml Bottle and Lid:2 ↔ Union Elbow 1-8 KQ2L01-00A SMC:11
- Mate:63: 40ml Bottle and Lid:2 ↔ Union Elbow 1-8 KQ2L01-00A SMC:12
- Mate:65: Internal Rear Plate:1 ↔ Battery Side Plate:1
- Flush:13: Top Divider:1 ↔ Battery Side Plate:1
- Mate:66: Top Divider:1 ↔ Battery Side Plate:1
- Mate:67 (0.1 mm): 22Ah BatteryPack:1 ↔ Battery Side Plate:1
- Flush:14: 22Ah BatteryPack:1 ↔ 22Ah BatteryPack:2
- Mate:69: Internal Rear Plate:1 ↔ Valve Assembly:1
- Mate:70: Port Support Plate:1 ↔ Mounted Pump:1
- Mate:72: Internal Rear Plate:1 ↔ Right Bracket 50mm RS749-1680:3
- Mate:73: Right Bracket 50mm RS749-1680:3 ↔ Top Divider:1
- Mate:74: Internal Rear Plate:1 ↔ Right Bracket 50mm RS749-1680:3
- Mate:75: Right Bracket 50mm RS749-1680:1 ↔ Inner Top Plate:1
- Mate:76: Right Bracket 50mm RS749-1680:2 ↔ Inner Top Plate:1
- Mate:77: Right Bracket 50mm RS749-1680:1 ↔ Inner Top Plate:1
- Mate:78: Enclosure RS746-7396 body:1 ↔ Vent Port M12:1
- Mate:79: Enclosure RS746-7396 body:1 ↔ Vent Port M12:2
- Mate:80: Enclosure RS746-7396 body:1 ↔ Vent Port M12:3
- Mate:81 (1 mm): Enclosure RS746-7396 body:1 ↔ Vent Port M12:2
- Mate:82 (1 mm): Enclosure RS746-7396 body:1 ↔ Vent Port M12:1
- Mate:83 (1 mm): Enclosure RS746-7396 body:1 ↔ Vent Port M12:3
- Mate:84: Enclosure RS746-7396 body:1 ↔ LED Indicator Assem Farnell 1368996:1
- Mate:85: Enclosure RS746-7396 body:1 ↔ LED Indicator Assem Farnell 1368996:3
- Mate:86: Enclosure RS746-7396 body:1 ↔ LED Indicator Assem Farnell 1368996:2
- Mate:87: Enclosure RS746-7396 body:1 ↔ LED Indicator Assem Farnell 1368996:2
- Mate:88: Enclosure RS746-7396 body:1 ↔ LED Indicator Assem Farnell 1368996:3
- Mate:89: Enclosure RS746-7396 body:1 ↔ LED Indicator Assem Farnell 1368996:1
- Mate:90: Enclosure RS746-7396 body:1 ↔ Omron Switch DigiKey_Z6183-NDA22NS_2B[]_N[]A_G[]00_NN:1
- Flush:15: Enclosure RS746-7396 body:1 ↔ Omron Switch DigiKey_Z6183-NDA22NS_2B[]_N[]A_G[]00_NN:1
- Angle:14 (0 deg): Top Divider:1 ↔ Omron Switch DigiKey_Z6183-NDA22NS_2B[]_N[]A_G[]00_NN:1
- Mate:91: Enclosure RS746-7396 body:1 ↔ Sprung Button Assm DigiKey EG5980-ND:1
- Mate:92: Enclosure RS746-7396 body:1 ↔ Sprung Button Assm DigiKey EG5980-ND:1
- Mate:94: Enclosure RS746-7396 body:1 ↔ Fixing Stud Pt 2:1
- Mate:96: Enclosure RS746-7396 body:1 ↔ Fixing Stud Pt 2:3
- Mate:97: Box Fixing Stud:1 ↔ Fixing Stud Pt 2:4
- Mate:98: Box Fixing Stud:1 ↔ Fixing Stud Pt 2:4
- Mate:99: Box Fixing Stud:3 ↔ Fixing Stud Pt 2:2
- Mate:100: Box Fixing Stud:4 ↔ Fixing Stud Pt 2:1
- Mate:101: Box Fixing Stud:3 ↔ Fixing Stud Pt 2:2
- Mate:102: Box Fixing Stud:2 ↔ Fixing Stud Pt 2:3
- Mate:103: Vent Port M12:1 ↔ Port Conversion Nut:1
- Mate:104: Vent Port M12:3 ↔ Port Conversion Nut:2
- Mate:105: Enclosure RS746-7396 body:1 ↔ M8 Mudguard Washer RS 660-4771:2
- Mate:106: Enclosure RS746-7396 body:1 ↔ M8 Mudguard Washer RS 660-4771:4
- Mate:107: Enclosure RS746-7396 body:1 ↔ M8 Mudguard Washer RS 660-4771:1
- Mate:108: Enclosure RS746-7396 body:1 ↔ M8 Mudguard Washer RS 660-4771:3
- Mate:109: Fixing Stud Pt 2:2 ↔ M8 Mudguard Washer RS 660-4771:3
- Mate:110: Fixing Stud Pt 2:3 ↔ M8 Mudguard Washer RS 660-4771:4
- Mate:111: Fixing Stud Pt 2:1 ↔ M8 Mudguard Washer RS 660-4771:2
- Mate:112: Fixing Stud Pt 2:4 ↔ M8 Mudguard Washer RS 660-4771:1
- Mate:113: Enclosure RS746-7396 body:1 ↔ M12 Tap washer RS 530-270:1
- Mate:114: Enclosure RS746-7396 body:1 ↔ M12 Tap washer RS 530-270:2
- Mate:115: Vent Port M12:3 ↔ M12 Tap washer RS 530-270:2
- Mate:116: Vent Port M12:1 ↔ M12 Tap washer RS 530-270:1
- Mate:117: M12 Form B A2 Washer RS 530-810:1 ↔ M12 Tap washer RS 530-270:1
- Mate:118: M12 Form B A2 Washer RS 530-810:2 ↔ M12 Tap washer RS 530-270:2
- Mate:119: Vent Port M12:3 ↔ M12 Form B A2 Washer RS 530-810:2
- Mate:120: Port Conversion Nut:2 ↔ M12 Form B A2 Washer RS 530-810:2
- Mate:121: Port Conversion Nut:1 ↔ M12 Form B A2 Washer RS 530-810:1
- Mate:122: Enclosure RS746-7396 body:1 ↔ Cable Gland Lock Nut RS 822-9791:1
- Mate:123: Vent Port M12:2 ↔ Cable Gland Lock Nut RS 822-9791:1
- Mate:124: Internal Rear Plate:1 ↔ Right Bracket 50mm RS749-1680:17
- Mate:125: Internal Rear Plate:1 ↔ Right Bracket 50mm RS749-1680:14
- Mate:126: Internal Rear Plate:1 ↔ Right Bracket 50mm RS749-1680:17
- Mate:127: Internal Rear Plate:1 ↔ Right Bracket 50mm RS749-1680:17
- Mate:128: Internal Rear Plate:1 ↔ Right Bracket 50mm RS749-1680:14
- Mate:129: Internal Rear Plate:1 ↔ Right Bracket 50mm RS749-1680:14
- Mate:130: Internal Rear Plate:1 ↔ Right Bracket 50mm RS749-1680:10
- Mate:131: Battery Side Plate:1 ↔ Right Bracket 50mm RS749-1680:10
- Mate:132: Battery Side Plate:1 ↔ Right Bracket 50mm RS749-1680:10
- Mate:133: Internal Rear Plate:1 ↔ Right Bracket 50mm RS749-1680:9
- Mate:134: Battery Side Plate:1 ↔ Right Bracket 50mm RS749-1680:9
- Mate:135: Battery Side Plate:1 ↔ Right Bracket 50mm RS749-1680:9
- Mate:136: Right Bracket 50mm RS749-1680:17 ↔ Battery Base Plate:1
- Mate:137: Right Bracket 50mm RS749-1680:14 ↔ Battery Base Plate:1
- Mate:138: Right Bracket 50mm RS749-1680:14 ↔ Battery Base Plate:1
- Mate:139: Internal Rear Plate:1 ↔ Right Bracket 50mm RS749-1680:13
- Mate:140: Internal Rear Plate:1 ↔ Right Bracket 50mm RS749-1680:13
- Mate:141: Internal Rear Plate:1 ↔ Right Bracket 50mm RS749-1680:13
- Mate:142: Right Bracket 50mm RS749-1680:13 ↔ Internal Vert Divider:1
- Mate:143: Right Bracket 50mm RS749-1680:13 ↔ Internal Vert Divider:1
- Mate:144: Right Bracket 50mm RS749-1680:13 ↔ Internal Vert Divider:1
- Mate:145: 22Ah BatteryPack:2 ↔ Battery Base Plate:1
- Flush:16: Union Elbow 1-8 KQ2L01-00A SMC:3 ↔ Union Elbow 1-8 KQ2L01-00A SMC:4
- Flush:17: Union Elbow 1-8 KQ2L01-00A SMC:11 ↔ Union Elbow 1-8 KQ2L01-00A SMC:12
- Flush:18: Union Elbow 1-8 KQ2L01-00A SMC:5 ↔ Union Elbow 1-8 KQ2L01-00A SMC:6
- Mate:157: Port Conversion Nut:1 ↔ M12 Form B A2 Washer RS 530-810:1
- Angle:16 (-90 deg): Internal Rear Plate:1 ↔ Union Elbow 1-8 KQ2L01-00A SMC:6
- Angle:17 (-90 deg): Internal Rear Plate:1 ↔ Union Elbow 1-8 KQ2L01-00A SMC:12
- Angle:18 (90 deg): Internal Rear Plate:1 ↔ Union Elbow 1-8 KQ2L01-00A SMC:3
- Mate:158: Port Conversion Nut:2 ↔ SMC10-32UNF-1-8 KQ2H01-32N RS 840-4665:2
- Mate:159: Port Conversion Nut:1 ↔ SMC10-32UNF-1-8 KQ2H01-32N RS 840-4665:1
- Mate:160: Port Conversion Nut:1 ↔ SMC10-32UNF-1-8 KQ2H01-32N RS 840-4665:1
- Mate:161: Port Conversion Nut:2 ↔ SMC10-32UNF-1-8 KQ2H01-32N RS 840-4665:2
- Mate:163: SMC10-32UNF-1-8 KQ2H01-32N RS 840-4665:1 ↔ Tube 1-8 5L:2
- Mate:164: SMC10-32UNF-1-8 KQ2H01-32N RS 840-4665:1 ↔ Tube 1-8 5L:2
- Mate:171: Union Elbow 1-8 KQ2L01-00A SMC:14 ↔ Union Elbow 1-8 KQ2L01-00A SMC:15
- Angle:21 (0 deg): Internal Rear Plate:1 ↔ Union Tee 1-8 KQ2T01-00A SMC:3
- Mate:174: Internal Rear Plate:1 ↔ Union Tee 1-8 KQ2T01-00A SMC:3
- Flush:20: 40ml Bottle and Lid:1 ↔ 40ml Bottle and Lid:4
- Flush:21: 40ml Bottle and Lid:1 ↔ 40ml Bottle and Lid:3
- Flush:22: 40ml Bottle and Lid:1 ↔ 40ml Bottle and Lid:2
- Angle:22 (0 deg): Internal Rear Plate:1 ↔ Union Elbow 1-8 KQ2L01-00A SMC:1
- Angle:23 (180 deg): Union Elbow 1-8 KQ2L01-00A SMC:9 ↔ Union Elbow 1-8 KQ2L01-00A SMC:14
- Angle:24 (180 deg): Internal Rear Plate:1 ↔ Union Elbow 1-8 KQ2L01-00A SMC:14
- Mate:176: Union Elbow 1-8 KQ2L01-00A SMC:9 ↔ Union Elbow 1-8 KQ2L01-00A SMC:14
- Mate:177: Internal Rear Plate:1 ↔ Union Elbow 1-8 KQ2L01-00A SMC:18
- Mate:178: Internal Rear Plate:1 ↔ Union Elbow 1-8 KQ2L01-00A SMC:2
- Mate:181: Union Elbow 1-8 KQ2L01-00A SMC:6 ↔ Union Tee 1-8 KQ2T01-00A SMC:3
- Flush:23: 40ml Bottle and Lid:4 ↔ 100ml Bottle and Lid:1
- Mate:182: Internal Rear Plate:1 ↔ Union Elbow 1-8 KQ2L01-00A SMC:1
- Mate:183: Internal Rear Plate:1 ↔ Union Elbow 1-8 KQ2L01-00A SMC:20
- Mate:184: Union Elbow 1-8 KQ2L01-00A SMC:5 ↔ Union Elbow 1-8 KQ2L01-00A SMC:20
- Mate:185: Union Elbow 1-8 KQ2L01-00A SMC:1 ↔ Union Elbow 1-8 KQ2L01-00A SMC:12
- Flush:24: Union Elbow 1-8 KQ2L01-00A SMC:1 ↔ Union Elbow 1-8 KQ2L01-00A SMC:20
- Angle:27 (0 deg): Internal Rear Plate:1 ↔ Union Elbow 1-8 KQ2L01-00A SMC:1
- Angle:28 (180 deg): Union Elbow 1-8 KQ2L01-00A SMC:5 ↔ Union Elbow 1-8 KQ2L01-00A SMC:20
- Angle:29 (0 deg): Internal Rear Plate:1 ↔ Union Tee 1-8 KQ2T01-00A SMC:2
- Mate:186: Internal Rear Plate:1 ↔ Union Tee 1-8 KQ2T01-00A SMC:2
- Mate:187: Union Elbow 1-8 KQ2L01-00A SMC:10 ↔ Union Tee 1-8 KQ2T01-00A SMC:2
- Mate:189: Union Tee 1-8 KQ2T01-00A SMC:2 ↔ Union Elbow 1-8 KQ2L01-00A SMC:16
- Mate:190 (5 mm): Union Tee 1-8 KQ2T01-00A SMC:2 ↔ Union Elbow 1-8 KQ2L01-00A SMC:16
- Mate:191: Internal Rear Plate:1 ↔ Valve Assembly:3
- Angle:32 (0 deg): Union Elbow 1-8 KQ2L01-00A SMC:5 ↔ Valve Assembly:3
- Mate:192 (5 mm): Union Elbow 1-8 KQ2L01-00A SMC:1 ↔ Union Elbow 1-8 KQ2L01-00A SMC:18
- Mate:193 (5 mm): Union Elbow 1-8 KQ2L01-00A SMC:20 ↔ Union Elbow 1-8 KQ2L01-00A SMC:21
- Mate:194: Union Elbow 1-8 KQ2L01-00A SMC:1 ↔ Union Elbow 1-8 KQ2L01-00A SMC:18
- Mate:195: Union Elbow 1-8 KQ2L01-00A SMC:20 ↔ Union Elbow 1-8 KQ2L01-00A SMC:21
- Mate:196: Internal Rear Plate:1 ↔ Valve Assembly:2
- Mate:197: Internal Rear Plate:1 ↔ Union Elbow 1-8 KQ2L01-00A SMC:17
- Angle:34 (180 deg): Valve Assembly:2 ↔ Valve Assembly:3
- Mate:199: Internal Rear Plate:1 ↔ Union Elbow 1-8 KQ2L01-00A SMC:19
- Mate:201: Union Elbow 1-8 KQ2L01-00A SMC:17 ↔ Union Elbow 1-8 KQ2L01-00A SMC:22
- Mate:202 (4 mm): Union Elbow 1-8 KQ2L01-00A SMC:19 ↔ Union Elbow 1-8 KQ2L01-00A SMC:22
- Mate:203: Union Elbow 1-8 KQ2L01-00A SMC:19 ↔ Union Elbow 1-8 KQ2L01-00A SMC:22
- Mate:204: Union Tee 1-8 KQ2T01-00A SMC:2 ↔ Union Tee 1-8 KQ2T01-00A SMC:3
- Flush:25: Union Elbow 1-8 KQ2L01-00A SMC:20 ↔ Union Elbow 1-8 KQ2L01-00A SMC:21
- Angle:35 (0 deg): Internal Rear Plate:1 ↔ Union Elbow 1-8 KQ2L01-00A SMC:17
- Angle:36 (180 deg): Internal Rear Plate:1 ↔ Union Elbow 1-8 KQ2L01-00A SMC:22
- Angle:37 (0 deg): Union Elbow 1-8 KQ2L01-00A SMC:22 ↔ Union Elbow 1-8 KQ2L01-00A SMC:26
- Mate:207: Union Elbow 1-8 KQ2L01-00A SMC:22 ↔ Union Elbow 1-8 KQ2L01-00A SMC:26
- Mate:208: Union Elbow 1-8 KQ2L01-00A SMC:24 ↔ Union Elbow 1-8 KQ2L01-00A SMC:26
- Mate:209: Union Elbow 1-8 KQ2L01-00A SMC:16 ↔ Union Elbow 1-8 KQ2L01-00A SMC:24
- Angle:38 (0 deg): Internal Rear Plate:1 ↔ Union Tee 1-8 KQ2T01-00A SMC:3
- Mate:210: Internal Rear Plate:1 ↔ Union Elbow 1-8 KQ2L01-00A SMC:23
- Mate:211: Union Elbow 1-8 KQ2L01-00A SMC:4 ↔ Union Elbow 1-8 KQ2L01-00A SMC:23
- Angle:39 (0 deg): Union Elbow 1-8 KQ2L01-00A SMC:17 ↔ Union Elbow 1-8 KQ2L01-00A SMC:23
- Angle:40 (0 deg): Valve Assembly:1 ↔ Valve Assembly:3
- Mate:221: Internal Rear Plate:1 ↔ Union Elbow 1-8 KQ2L01-00A SMC:28
- Mate:222: Internal Rear Plate:1 ↔ Union Elbow 1-8 KQ2L01-00A SMC:29
- Mate:223: Union Elbow 1-8 KQ2L01-00A SMC:7 ↔ Union Elbow 1-8 KQ2L01-00A SMC:29
- Mate:224: Internal Rear Plate:1 ↔ Union Elbow 1-8 KQ2L01-00A SMC:30
- Mate:226 (75 mm): Union Elbow 1-8 KQ2L01-00A SMC:28 ↔ Union Elbow 1-8 KQ2L01-00A SMC:29
- Angle:44 (0 deg): Union Elbow 1-8 KQ2L01-00A SMC:20 ↔ Union Elbow 1-8 KQ2L01-00A SMC:29
- Mate:227: Internal Rear Plate:1 ↔ Union Elbow 1-8 KQ2L01-00A SMC:31
- Mate:229: Full Cartridge Interface:1 ↔ Legris4-4mm Elbow 31820400 RS 306-5993:2
- Mate:230: Full Cartridge Interface:1 ↔ Legris4-4mm Elbow 31820400 RS 306-5993:2
- Mate:231: Full Cartridge Interface:1 ↔ Legris4-4mm Elbow 31820400 RS 306-5993:1
- Mate:232: Full Cartridge Interface:1 ↔ Legris4-4mm Elbow 31820400 RS 306-5993:1
- Angle:45 (180 deg): Top Divider:1 ↔ Legris4-4mm Elbow 31820400 RS 306-5993:1
- Angle:46 (180 deg): Top Divider:1 ↔ Legris4-4mm Elbow 31820400 RS 306-5993:2
- Angle:47 (180 deg): Top Divider:1 ↔ Union Elbow 1-8 KQ2L01-00A SMC:34
- Angle:48 (180 deg): Internal Rear Plate:1 ↔ Union Elbow 1-8 KQ2L01-00A SMC:34
- Mate:233 (30 mm): Top Divider:1 ↔ Union Elbow 1-8 KQ2L01-00A SMC:34
- Mate:234: Legris4-4mm Elbow 31820400 RS 306-5993:2 ↔ Union Elbow 1-8 KQ2L01-00A SMC:34
- Mate:235: Internal Rear Plate:1 ↔ Union Elbow 1-8 KQ2L01-00A SMC:33
- Mate:236: Union Elbow 1-8 KQ2L01-00A SMC:33 ↔ Union Elbow 1-8 KQ2L01-00A SMC:34
- Angle:49 (0 deg): Union Elbow 1-8 KQ2L01-00A SMC:19 ↔ Union Elbow 1-8 KQ2L01-00A SMC:33
- Mate:238: Internal Rear Plate:1 ↔ Union Elbow 1-8 KQ2L01-00A SMC:35
- Mate:239 (48 mm): Union Tee 1-8 KQ2T01-00A SMC:1 ↔ Union Elbow 1-8 KQ2L01-00A SMC:35
- Mate:240: Union Tee 1-8 KQ2T01-00A SMC:1 ↔ Union Elbow 1-8 KQ2L01-00A SMC:35
- Angle:50 (180 deg): Union Tee 1-8 KQ2T01-00A SMC:1 ↔ Union Elbow 1-8 KQ2L01-00A SMC:30
- Angle:51 (0 deg): Union Elbow 1-8 KQ2L01-00A SMC:29 ↔ Union Elbow 1-8 KQ2L01-00A SMC:30
- Mate:241: Union Tee 1-8 KQ2T01-00A SMC:1 ↔ Union Elbow 1-8 KQ2L01-00A SMC:33
- Mate:242: Legris4-4mm Elbow 31820400 RS 306-5993:2 ↔ SMC 4mmMale-1-8Push KQ2R01-03(R23-04):2
- Flush:26 (-18 mm): Legris4-4mm Elbow 31820400 RS 306-5993:2 ↔ SMC 4mmMale-1-8Push KQ2R01-03(R23-04):2
- Mate:243: Legris4-4mm Elbow 31820400 RS 306-5993:1 ↔ SMC Nipple 1-8to5-32 KQ2N01-03:1
- Flush:27 (26.5 mm): Legris4-4mm Elbow 31820400 RS 306-5993:1 ↔ SMC Nipple 1-8to5-32 KQ2N01-03:1
- Mate:244 (15 mm): Top Divider:1 ↔ SMC AS2002F Needle Valve RS 827-0755:1
- Mate:246: SMC AS2002F Needle Valve RS 827-0755:1 ↔ SMC Nipple 1-8to5-32 KQ2N01-03:2
- Flush:28 (-26 mm): SMC AS2002F Needle Valve RS 827-0755:1 ↔ SMC Nipple 1-8to5-32 KQ2N01-03:2
- Mate:248 (-10 mm): SMC AS2002F Needle Valve RS 827-0755:1 ↔ SMC Elbow KQ2L23-04:2
- Mate:251: SMC10-32UNF-1-8 KQ2H01-32N RS 840-4665:1 ↔ Union Elbow 1-8 KQ2L01-00A SMC:32
- Mate:252: SMC AS2002F Needle Valve RS 827-0755:1 ↔ SMC Elbow KQ2L23-04:2
- Mate:253: Right Bracket 30mm RS749-1686:8 ↔ Union Elbow 1-8 KQ2L01-00A SMC:32
- Mate:254: Right Bracket 30mm RS749-1686:8 ↔ Union Elbow 1-8 KQ2L01-00A SMC:32
- Mate:255: Right Bracket 30mm RS749-1686:8 ↔ Internal Vert Divider:1
- Angle:53 (0 deg): Internal Rear Plate:1 ↔ Union Elbow 1-8 KQ2L01-00A SMC:28
- Mate:256 (34 mm): Union Elbow 1-8 KQ2L01-00A SMC:9 ↔ Union Elbow 1-8 KQ2L01-00A SMC:14
- Mate:257: Internal Rear Plate:1 ↔ Bottle Base Plate:1
- Mate:258: Internal Vert Divider:1 ↔ Bottle Base Plate:1
- Mate:268: 100ml Bottle and Lid:1 ↔ Bottle Base Plate:1
- Mate:269: Internal Rear Plate:1 ↔ No Thrd Right Support Farnell1466881:1
- Mate:270: Internal Rear Plate:1 ↔ No Thrd Right Support Farnell1466881:2
- Mate:271: Internal Vert Divider:1 ↔ No Thrd Right Support Farnell1466881:3
- Mate:272: Internal Vert Divider:1 ↔ No Thrd Right Support Farnell1466881:9
- Mate:273: Internal Rear Plate:1 ↔ No Thrd Right Support Farnell1466881:1
- Mate:274: Internal Rear Plate:1 ↔ No Thrd Right Support Farnell1466881:2
- Mate:275: Bottle Base Plate:1 ↔ No Thrd Right Support Farnell1466881:1
- Mate:276: Bottle Base Plate:1 ↔ No Thrd Right Support Farnell1466881:2
- Angle:54 (0 deg): Right Bracket 30mm RS749-1686:8 ↔ Union Elbow 1-8 KQ2L01-00A SMC:32
- Mate:277: Union Elbow 1-8 KQ2L01-00A SMC:23 ↔ Union Elbow 1-8 KQ2L01-00A SMC:31
- Angle:55 (0 deg): Union Tee 1-8 KQ2T01-00A SMC:1 ↔ Union Elbow 1-8 KQ2L01-00A SMC:28
- Angle:56 (180 deg): Internal Rear Plate:1 ↔ Cable Clip 3-1Dia RS817-8956:2
- Angle:57 (180 deg): Internal Rear Plate:1 ↔ Cable Clip 3-1Dia RS817-8956:4
- Angle:58 (180 deg): Internal Rear Plate:1 ↔ Cable Clip 3-1Dia RS817-8956:3
- Mate:278: Union Elbow 1-8 KQ2L01-00A SMC:35 ↔ Cable Clip 3-1Dia RS817-8956:2
- Mate:279: Union Elbow 1-8 KQ2L01-00A SMC:35 ↔ Cable Clip 3-1Dia RS817-8956:4
- Mate:280: Union Elbow 1-8 KQ2L01-00A SMC:35 ↔ Cable Clip 3-1Dia RS817-8956:4
- Mate:281: Union Elbow 1-8 KQ2L01-00A SMC:35 ↔ Cable Clip 3-1Dia RS817-8956:2
- Mate:282: Union Elbow 1-8 KQ2L01-00A SMC:28 ↔ Cable Clip 3-1Dia RS817-8956:5
- Mate:283: Union Elbow 1-8 KQ2L01-00A SMC:28 ↔ Cable Clip 3-1Dia RS817-8956:6
- Mate:284: Union Elbow 1-8 KQ2L01-00A SMC:28 ↔ Cable Clip 3-1Dia RS817-8956:6
- Mate:285: Union Elbow 1-8 KQ2L01-00A SMC:28 ↔ Cable Clip 3-1Dia RS817-8956:5
- Mate:290: Union Elbow 1-8 KQ2L01-00A SMC:26 ↔ Cable Clip 3-1Dia RS817-8956:9
- Mate:291: Union Elbow 1-8 KQ2L01-00A SMC:26 ↔ Cable Clip 3-1Dia RS817-8956:9
- Mate:292: Internal Rear Plate:1 ↔ Union Elbow 1-8 KQ2L01-00A SMC:26
- Mate:295: Union Elbow 1-8 KQ2L01-00A SMC:19 ↔ Cable Clip 3-1Dia RS817-8956:12
- Mate:296: Union Elbow 1-8 KQ2L01-00A SMC:19 ↔ Cable Clip 3-1Dia RS817-8956:12
- Mate:299: Union Elbow 1-8 KQ2L01-00A SMC:33 ↔ Cable Clip 3-1Dia RS817-8956:13
- Mate:300: Union Elbow 1-8 KQ2L01-00A SMC:33 ↔ Cable Clip 3-1Dia RS817-8956:13